# Autodesk Inventor assembly: Butterfly Drive Module
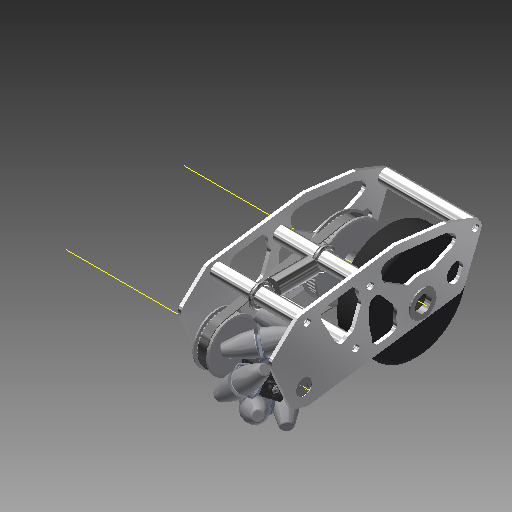
[picture p0: Inventor's stored thumbnail of the model, 512x512]
Saved by Autodesk Inventor 2019 (Build 230136000, 136)
## iProperties
Created: 2019-11-02
Part Number: Butterfly Drive Module
Document SubType Name: Assembly
Designer: admin
Mass: 2776.16 g
Surface Area: 3944.64 cm^2
Volume: 1383.77 cm^3
Density: 2.00623 g/cm^3
Author: admin
## Documents named in this file (13)
- C:\Users\Mark\Desktop\7738 Helion Engineering\7738-CAD-prep\Butterfly Drive Mk2\Butterfly Module\Butterfly Drive Module.iam
- C:\Users\Mark\Desktop\7738 Helion Engineering\7738-CAD-prep\Butterfly Drive Mk2\Butterfly Module\100mm Mecanum StandIn.ipt
- C:\Users\Mark\Desktop\7738 Helion Engineering\7738-CAD-prep\Butterfly Drive Mk2\Butterfly Module\100mm Traction Wheel StandIn.ipt
- C:\Users\Mark\Desktop\7738 Helion Engineering\7738-CAD-prep\Butterfly Drive Mk2\Butterfly Module\Connector.ipt
- C:\Users\Mark\Desktop\7738 Helion Engineering\7738-CAD-prep\Butterfly Drive Mk2\Butterfly Module\M6GBTeye.ipt
- C:\Users\Mark\Desktop\7738 Helion Engineering\7738-CAD-prep\Butterfly Drive Mk2\Butterfly Module\Module Plate 1.ipt
- C:\Users\Mark\Desktop\7738 Helion Engineering\7738-CAD-prep\Butterfly Drive Mk2\Butterfly Module\Butterfly Drive Module\Design Accelerator\Synchronous Belts Transmission1.iam
- C:\Users\Mark\Desktop\7738 Helion Engineering\7738-CAD-prep\Butterfly Drive Mk2\Butterfly Module\Pneumatics Connector.ipt
- C:\Users\Mark\Desktop\7738 Helion Engineering\7738-CAD-prep\Butterfly Drive Mk2\Butterfly Module\F6004.ipt
- C:\Users\Mark\Desktop\7738 Helion Engineering\7738-CAD-prep\Butterfly Drive Mk2\Butterfly Module\Mecanum Axle.ipt
- C:\Users\Mark\Desktop\7738 Helion Engineering\7738-CAD-prep\Butterfly Drive Mk2\Butterfly Module\Butterfly Drive Module\Design Accelerator\Key Connection1.iam
- C:\Users\Mark\Desktop\7738 Helion Engineering\7738-CAD-prep\Butterfly Drive Mk2\Butterfly Base\F6800Z 10mm ID Flange.ipt
- C:\Users\Mark\Desktop\7738 Helion Engineering\7738-CAD-prep\Butterfly Drive Mk2\Butterfly Base\4_Mecanum_Wheel_Left_217-3644.iam
## Components (19 placed, 12 different names)
1. 100mm Mecanum StandIn:1 — Mate:2, Flush:1, Mate:19, Angle:1
2. 100mm Traction Wheel StandIn:1 — Flush:1, Mate:50, Mate:64
3. Connector:1 — Mate:5, Mate:6, Mate:10, Mate:44
4. M6GBTeye:1 — Mate:9, Mate:11, Mate:33
5. Module Plate 1:1 — Mate:2, Mate:5, Mate:6, Mate:7, Mate:8, Mate:37, Mate:38, Mate:39, Mate:40, Mate:41, Mate:51, Angle:2, Mate:56, Mate:57, Mate:59
6. Connector:2 — Mate:7, Mate:8, Mate:9
7. M6GBTeye:2 — Mate:10, Mate:11, Flush:3
8. Synchronous Belts Transmission:1 [sub-assembly] — Mate:19, Mate:28, Mate:29, Mate:31, Angle:1, Mate:50, Angle:2, Mate:59, Mate:60
9. Pneumatics Connector:1 — Mate:33, Flush:3, Mate:49
10. F6004:2 — Mate:37, Mate:51
11. Connector:3 — Mate:38, Mate:39, Mate:45, Mate:46
12. Connector:4 — Mate:40, Mate:41
13. Mecanum Axle:1 — Mate:53, Mate:55, Flush:5, Mate:58, Mate:61, Mate:62, Mate:63
14. Key Connection:1 [sub-assembly]
15. Module Plate 1:2 — Mate:44, Mate:45, Mate:46, Mate:48, Mate:49
16. F6004:3 — Mate:48, Mate:64
17. F6800Z 10mm ID Flange:1 — Mate:62, Mate:63
18. 4_Mecanum_Wheel_Left_217-3644:1 [sub-assembly] — Mate:53, Mate:55, Flush:5
19. F6800Z 10mm ID Flange:2 — Mate:56, Mate:57, Mate:58, Mate:60, Mate:61
## Relationships (45: Mate 40, Flush 3, Angle 2)
- Mate:2: 100mm Mecanum StandIn:1 ↔ Module Plate 1:1
- Mate:5: Connector:1 ↔ Module Plate 1:1
- Mate:6 (0.3 mm): Connector:1 ↔ Module Plate 1:1
- Mate:7: Module Plate 1:1 ↔ Connector:2
- Mate:8 (0.3 mm): Module Plate 1:1 ↔ Connector:2
- Mate:9: M6GBTeye:1 ↔ Connector:2
- Mate:10: Connector:1 ↔ M6GBTeye:2
- Mate:11: M6GBTeye:1 ↔ M6GBTeye:2
- Flush:1: 100mm Mecanum StandIn:1 ↔ 100mm Traction Wheel StandIn:1
- Mate:14
- Mate:15
- Mate:19 (3 mm): 100mm Mecanum StandIn:1 ↔ Synchronous Belts Transmission:1
- Mate:28: Synchronous Belts Transmission:1
- Mate:29: Synchronous Belts Transmission:1
- Mate:30
- Mate:31: Synchronous Belts Transmission:1
- Mate:32
- Mate:33: M6GBTeye:1 ↔ Pneumatics Connector:1
- Flush:3 (2 mm): M6GBTeye:2 ↔ Pneumatics Connector:1
- Mate:37 (0.3 mm): Module Plate 1:1 ↔ F6004:2
- Mate:38: Module Plate 1:1 ↔ Connector:3
- Mate:39 (0.3 mm): Module Plate 1:1 ↔ Connector:3
- Mate:40: Module Plate 1:1 ↔ Connector:4
- Mate:41 (0.3 mm): Module Plate 1:1 ↔ Connector:4
- Angle:1 (0 deg): 100mm Mecanum StandIn:1 ↔ Synchronous Belts Transmission:1
- Mate:44: Connector:1 ↔ Module Plate 1:2
- Mate:45: Connector:3 ↔ Module Plate 1:2
- Mate:46 (0.3 mm): Connector:3 ↔ Module Plate 1:2
- Mate:48 (0.3 mm): Module Plate 1:2 ↔ F6004:3
- Mate:49 (52.5 mm): Pneumatics Connector:1 ↔ Module Plate 1:2
- Mate:50: 100mm Traction Wheel StandIn:1 ↔ Synchronous Belts Transmission:1
- Mate:51: Module Plate 1:1 ↔ F6004:2
- Angle:2 (-3.25 deg): Module Plate 1:1 ↔ Synchronous Belts Transmission:1
- Mate:53: Mecanum Axle:1 ↔ 4_Mecanum_Wheel_Left_217-3644:1
- Mate:55: Mecanum Axle:1 ↔ 4_Mecanum_Wheel_Left_217-3644:1
- Flush:5: Mecanum Axle:1 ↔ 4_Mecanum_Wheel_Left_217-3644:1
- Mate:56: Module Plate 1:1 ↔ F6800Z 10mm ID Flange:2
- Mate:57 (0.3 mm): Module Plate 1:1 ↔ F6800Z 10mm ID Flange:2
- Mate:58: Mecanum Axle:1 ↔ F6800Z 10mm ID Flange:2
- Mate:59 (5 mm): Module Plate 1:1 ↔ Synchronous Belts Transmission:1
- Mate:60: Synchronous Belts Transmission:1 ↔ F6800Z 10mm ID Flange:2
- Mate:61 (0.3 mm): Mecanum Axle:1 ↔ F6800Z 10mm ID Flange:2
- Mate:62: Mecanum Axle:1 ↔ F6800Z 10mm ID Flange:1
- Mate:63 (0.3 mm): Mecanum Axle:1 ↔ F6800Z 10mm ID Flange:1
- Mate:64: 100mm Traction Wheel StandIn:1 ↔ F6004:3
